# Autodesk Inventor assembly: Дверка
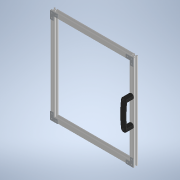
[picture p0: Inventor's stored thumbnail of the model, 180x180]
Saved by Autodesk Inventor 2020 (Build 240168000, 168)
## iProperties
Created: 2020-04-03
Part Number: Дверка
Document SubType Name: Assembly
Designer: Михаил
Author: Михаил
## Documents named in this file (5)
- D:\MyWorks\GrowBox_v2\3D_body\Дверка.iam
- D:\MyWorks\GrowBox_v2\3D_body\G_soedinitel-40x40.ipt
- D:\MyWorks\GrowBox_v2\3D_body\Профиль_аллюминиевый355.ipt
- D:\MyWorks\GrowBox_v2\3D_body\Профиль_аллюминиевый450.ipt
- D:\MyWorks\GrowBox_v2\3D_body\Ruchka-dvernaya-plastikovaya_-120mm_T10_.ipt
## Components (9 placed, 3 different names)
1. G_soedinitel-40x40:1 — Заподлицо:10, Совмещение:5, Заподлицо:11
2. Профиль_алюминиевый:1 — Совмещение:1, Заподлицо:1, Заподлицо:2, Совмещение:5, Заподлицо:11
3. Профиль_алюминиевый:2 — Совмещение:1, Заподлицо:1, Заподлицо:2, Совмещение:2, Заподлицо:3, Заподлицо:4, Совмещение:4, Заподлицо:7, Заподлицо:8, Совмещение:6, Заподлицо:13
4. G_soedinitel-40x40:2 — Совмещение:4, Заподлицо:7, Заподлицо:8
5. Профиль_алюминиевый:3 — Совмещение:2, Заподлицо:3, Заподлицо:4, Заподлицо:5, Совмещение:3, Заподлицо:6, Заподлицо:12
6. Профиль_алюминиевый:4 — Заподлицо:5, Совмещение:3, Заподлицо:6, Заподлицо:10, Совмещение:7, Заподлицо:14, Заподлицо:15, Совмещение:8
7. G_soedinitel-40x40:3 — Совмещение:6, Заподлицо:12, Заподлицо:13
8. G_soedinitel-40x40:4 — Совмещение:7, Заподлицо:14, Заподлицо:15
9. Ruchka-dvernaya-plastikovaya_-120mm_T10_:1 — Совмещение:8
## Relationships (22: Flush 14, Mate 8)
- Совмещение:1 [Mate]: Профиль_алюминиевый:1 ↔ Профиль_алюминиевый:2
- Заподлицо:1 [Flush]: Профиль_алюминиевый:1 ↔ Профиль_алюминиевый:2
- Заподлицо:2 [Flush]: Профиль_алюминиевый:1 ↔ Профиль_алюминиевый:2
- Совмещение:2 [Mate]: Профиль_алюминиевый:2 ↔ Профиль_алюминиевый:3
- Заподлицо:3 [Flush]: Профиль_алюминиевый:2 ↔ Профиль_алюминиевый:3
- Заподлицо:4 [Flush]: Профиль_алюминиевый:2 ↔ Профиль_алюминиевый:3
- Заподлицо:5 [Flush]: Профиль_алюминиевый:3 ↔ Профиль_алюминиевый:4
- Совмещение:3 [Mate]: Профиль_алюминиевый:3 ↔ Профиль_алюминиевый:4
- Заподлицо:6 [Flush]: Профиль_алюминиевый:3 ↔ Профиль_алюминиевый:4
- Совмещение:4 [Mate]: Профиль_алюминиевый:2 ↔ G_soedinitel-40x40:2
- Заподлицо:7 [Flush]: Профиль_алюминиевый:2 ↔ G_soedinitel-40x40:2
- Заподлицо:8 [Flush]: Профиль_алюминиевый:2 ↔ G_soedinitel-40x40:2
- Заподлицо:10 [Flush]: G_soedinitel-40x40:1 ↔ Профиль_алюминиевый:4
- Совмещение:5 [Mate]: G_soedinitel-40x40:1 ↔ Профиль_алюминиевый:1
- Заподлицо:11 [Flush]: G_soedinitel-40x40:1 ↔ Профиль_алюминиевый:1
- Совмещение:6 [Mate]: Профиль_алюминиевый:2 ↔ G_soedinitel-40x40:3
- Заподлицо:12 [Flush]: Профиль_алюминиевый:3 ↔ G_soedinitel-40x40:3
- Заподлицо:13 [Flush]: Профиль_алюминиевый:2 ↔ G_soedinitel-40x40:3
- Совмещение:7 [Mate]: Профиль_алюминиевый:4 ↔ G_soedinitel-40x40:4
- Заподлицо:14 [Flush]: Профиль_алюминиевый:4 ↔ G_soedinitel-40x40:4
- Заподлицо:15 [Flush]: Профиль_алюминиевый:4 ↔ G_soedinitel-40x40:4
- Совмещение:8 [Mate]: Профиль_алюминиевый:4 ↔ Ruchka-dvernaya-plastikovaya_-120mm_T10_:1
